# Autodesk Inventor assembly: Montaje
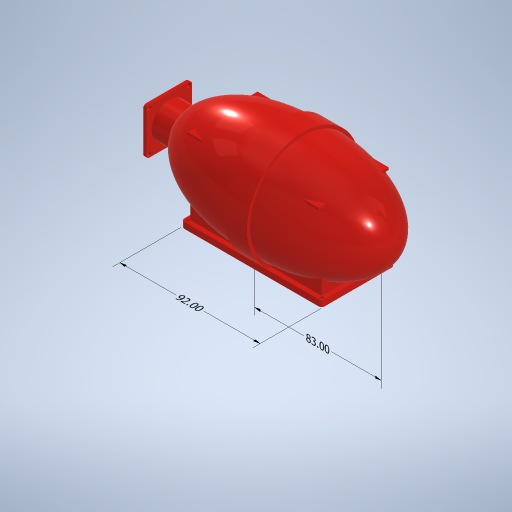
[picture p0: Inventor's stored thumbnail of the model, 512x512]
Saved by Autodesk Inventor 2023 (Build 270158000, 158)
## iProperties
Created: 2023-03-28
Part Number: Montaje
Document SubType Name: Assembly
Designer: andre
Author: andre
## Documents named in this file (3)
- C:\Users\andre\OneDrive\Desktop\Final jobb\Montaje.iam
- C:\Users\andre\OneDrive\Desktop\Final jobb\Estructura1.ipt
- C:\Users\andre\OneDrive\Desktop\Final jobb\Estructura2.ipt
## Components (2 placed, 2 different names)
1. Estructura1:1 — Rigid:1
2. Estructura2:1 — Rigid:1
## Relationships (1: WeldJoint 1)
- Rigid:1 [WeldJoint]: Estructura1:1 ↔ Estructura2:1
